# Autodesk Inventor assembly: Łodyga.ipt
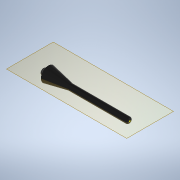
[picture p0: Inventor's stored thumbnail of the model, 180x180]
Saved by Autodesk Inventor 2022 (Build 260153000, 153)
## iProperties
Created: 2023-04-14
Part Number: Łodyga.ipt
Document SubType Name: Assembly
Designer: Szymon Chmielewski
Author: Szymon Chmielewski
## Documents named in this file (2)
- C:\Users\Szymon Chmielewski\Desktop\NAUKA\STUDIA\SEMESTR 6\Implanty\Łodyga.ipt.iam
- C:\Users\Szymon Chmielewski\Documents\Inventor\Shaft3.ipt
## Components (1 placed, 1 different names)
1. Shaft:1
## Relationships (1: Flush 1)
- Flush:1 (18.25 mm)
